# Autodesk Inventor assembly: dome one terminal
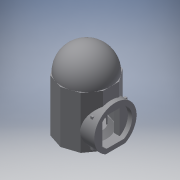
[picture p0: Inventor's stored thumbnail of the model, 180x180]
Saved by Autodesk Inventor 2017 (Build 210142000, 142)
## iProperties
Created: 2018-04-12
Part Number: dome one terminal
Document SubType Name: Assembly
Designer: Braxton
Author: Braxton
## Documents named in this file (4)
- E:\School\Game develpment\geoscape\done\rooms\assembly\dome one terminal.iam
- E:\School\Game develpment\geoscape\done\rooms\dome one terminal.ipt
- E:\School\Game develpment\geoscape\done\terminal\terminal assembly with railings.iam
- E:\School\Game develpment\geoscape\done\doors\double door.ipt
## Components (4 placed, 3 different names)
1. dome one terminal:1 — Flush:1, Mate:1, Mate:2, Mate:3, Mate:4, Mate:5, Mate:6, Mate:7, Mate:8
2. terminal assembly with railings:1 [sub-assembly] — Flush:1, Mate:1, Mate:2
3. double door:1 — Mate:3, Mate:6, Mate:7
4. double door:2 — Mate:4, Mate:5, Mate:8
## Relationships (9: Mate 8, Flush 1)
- Flush:1: dome one terminal:1 ↔ terminal assembly with railings:1
- Mate:1: dome one terminal:1 ↔ terminal assembly with railings:1
- Mate:2 (119.1705 mm): dome one terminal:1 ↔ terminal assembly with railings:1
- Mate:3: dome one terminal:1 ↔ double door:1
- Mate:4: dome one terminal:1 ↔ double door:2
- Mate:5: dome one terminal:1 ↔ double door:2
- Mate:6: dome one terminal:1 ↔ double door:1
- Mate:7: dome one terminal:1 ↔ double door:1
- Mate:8: dome one terminal:1 ↔ double door:2
